# Autodesk Inventor assembly: 74. Вал первичный в сборе
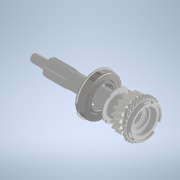
[picture p0: Inventor's stored thumbnail of the model, 180x180]
Saved by Autodesk Inventor 2021 (Build 250183000, 183)
## iProperties
Created: 2021-04-05
Part Number: 74. Вал первичный в сборе
Document SubType Name: Assembly
Designer: Данил
Author: Данил
## Documents named in this file (8)
- C:\Users\Данил\Desktop\Коробка передач\Детали\74. Вал первичный в сборе.iam
- C:\Users\Данил\Desktop\Коробка передач\Детали\74. Комплект первичного вала с кольцом после притирки.iam
- C:\Users\Данил\Desktop\Коробка передач\Детали\76. Гайка первичного вала.ipt
- C:\Users\Данил\Desktop\Коробка передач\Детали\65. Кольцо упорное подшипника.ipt
- C:\Users\Данил\Desktop\Коробка передач\Детали\68. Шайба упорная.ipt
- C:\Users\Данил\Desktop\Коробка передач\Детали\68. Кольцо стопорное подшипника.ipt
- C:\Users\Данил\Desktop\Коробка передач\Детали\74. Ролик вала.ipt
- C:\Users\Данил\Desktop\Коробка передач\Детали\Подшипник 180209 ГОСТ 8882-75.ipt
## Components (20 placed, 7 different names)
1. 74. Комплект первичного вала с кольцом после притирки:1 [sub-assembly] — Совмещение:1, Совмещение:9, Касательность:1, Совмещение:11, Совмещение:13, Совмещение:14, Совмещение:15, Совмещение:18
2. 76. Гайка первичного вала:1 — Совмещение:1, Совмещение:19
3. 65. Кольцо упорное подшипника:1 — Совмещение:16, Совмещение:17
4. 68. Шайба упорная:1 — Совмещение:11, Совмещение:12
5. 68. Кольцо стопорное подшипника:1 — Совмещение:13, Совмещение:14
6. Подшипник 180000 ГОСТ 8882-75 180209:1 — Совмещение:15, Совмещение:16, Совмещение:17, Совмещение:18, Совмещение:19
7. 74. Ролик вала:1 — Совмещение:9, Совмещение:10, Касательность:1
8. 74. Ролик вала:2
9. 74. Ролик вала:3 — Совмещение:12
10. 74. Ролик вала:4
11. 74. Ролик вала:5
12. 74. Ролик вала:6
13. 74. Ролик вала:7
14. 74. Ролик вала:8
15. 74. Ролик вала:9
16. 74. Ролик вала:10
17. 74. Ролик вала:11
18. 74. Ролик вала:12
19. 74. Ролик вала:13
20. 74. Ролик вала:14
## Component patterns: (14 elements, first: 74. Ролик вала:1)
## Relationships (13: Mate 12, Tangent 1)
- Совмещение:1 [Mate]: 74. Комплект первичного вала с кольцом после притирки:1 ↔ 76. Гайка первичного вала:1
- Совмещение:9 [Mate]: 74. Комплект первичного вала с кольцом после притирки:1 ↔ 74. Ролик вала:1
- Совмещение:10 [Mate]: 74. Ролик вала:1
- Касательность:1 [Tangent]: 74. Комплект первичного вала с кольцом после притирки:1 ↔ 74. Ролик вала:1
- Совмещение:11 [Mate]: 74. Комплект первичного вала с кольцом после притирки:1 ↔ 68. Шайба упорная:1
- Совмещение:12 [Mate]: 68. Шайба упорная:1 ↔ 74. Ролик вала:3
- Совмещение:13 [Mate]: 74. Комплект первичного вала с кольцом после притирки:1 ↔ 68. Кольцо стопорное подшипника:1
- Совмещение:14 [Mate]: 74. Комплект первичного вала с кольцом после притирки:1 ↔ 68. Кольцо стопорное подшипника:1
- Совмещение:15 [Mate]: 74. Комплект первичного вала с кольцом после притирки:1 ↔ Подшипник 180000 ГОСТ 8882-75 180209:1
- Совмещение:16 [Mate]: 65. Кольцо упорное подшипника:1 ↔ Подшипник 180000 ГОСТ 8882-75 180209:1
- Совмещение:17 [Mate]: 65. Кольцо упорное подшипника:1 ↔ Подшипник 180000 ГОСТ 8882-75 180209:1
- Совмещение:18 [Mate]: 74. Комплект первичного вала с кольцом после притирки:1 ↔ Подшипник 180000 ГОСТ 8882-75 180209:1
- Совмещение:19 [Mate]: 76. Гайка первичного вала:1 ↔ Подшипник 180000 ГОСТ 8882-75 180209:1
